# Autodesk Inventor assembly: センサ2個積み
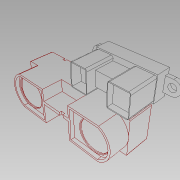
[picture p0: Inventor's stored thumbnail of the model, 180x180]
Saved by Autodesk Inventor 2017 (Build 210142000, 142)
## iProperties
Part Number: センサ2個積み
Material: 一般
Document SubType Name: Assembly
Designer: HISAAKI
Author: HISAAKI
## Documents named in this file (3)
- C:\Users\HISAAKI\Documents\LYNCS\CanSat\2017種子島\cansat-structure\センサ2個積み.iam
- C:\Users\HISAAKI\Documents\LYNCS\CanSat\2017種子島\cansat-structure\Sharp_2Y0A710.ipt
- C:\Users\HISAAKI\Documents\LYNCS\CanSat\2017種子島\cansat-structure\SharpDistanceRanger.ipt
## Components (2 placed, 2 different names)
1. Sharp_2Y0A710:1 — メイト:1, フラッシュ:1, メイト:2
2. SharpDistanceRanger:1 — メイト:1, フラッシュ:1, メイト:2
## Relationships (3: Mate 2, Flush 1)
- メイト:1 [Mate]: Sharp_2Y0A710:1 ↔ SharpDistanceRanger:1
- フラッシュ:1 [Flush]: Sharp_2Y0A710:1 ↔ SharpDistanceRanger:1
- メイト:2 [Mate]: Sharp_2Y0A710:1 ↔ SharpDistanceRanger:1
